# Autodesk Inventor assembly: DriveShaftA
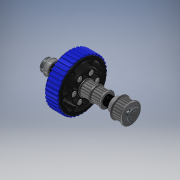
[picture p0: Inventor's stored thumbnail of the model, 180x180]
Saved by Autodesk Inventor 2018 (Build 220112000, 112)
## iProperties
Created: 2017-09-03
Part Number: DriveShaftA
Document SubType Name: Assembly
Designer: snipe
Author: snipe
## Documents named in this file (10)
- E:\Clark\Assets\DriveShaftA.iam
- E:\Clark\Assets\ThunderHex_DriveShaft.ipt
- E:\Clark\Assets\FlangedThunderHexBearing.ipt
- E:\Clark\Assets\ShaftCollar.ipt
- E:\Clark\Assets\0.5inSpacer.ipt
- E:\Clark\Assets\0.25inSpacer.ipt
- E:\Clark\Assets\0.125inSpacer.ipt
- E:\Clark\Assets\18tPulley15mm.ipt
- E:\Clark\Assets\PlactionWheelwithHubnoBearing.iam
- E:\Clark\Assets\24tPulley15mm.ipt
## Components (15 placed, 9 different names)
1. ThunderHex_DriveShaft:1 — Flush:1, Mate:1, Mate:2, Mate:4, Mate:5, Mate:7, Mate:9, Mate:10, Mate:12, Mate:13, Mate:15, Mate:16, Mate:18, Mate:19, Mate:21, Mate:22, Mate:24, Mate:25, Mate:27, Mate:28, Mate:30, Mate:32, Mate:33, Mate:35, Mate:36, Mate:38, Mate:39
2. FlangedThunderHexBearing:1 — Mate:29, Mate:30, Mate:31
3. FlangedThunderHexBearing:2 — Mate:6, Mate:7, Mate:8
4. ShaftCollar:1 — Flush:1, Mate:1, Mate:2, Mate:3
5. ShaftCollar:2 — Mate:35, Mate:36, Mate:40
6. 0.5inSpacer:1 — Mate:8, Mate:9, Mate:10, Mate:11
7. 0.5inSpacer:2 — Mate:23, Mate:24, Mate:25, Mate:26
8. 0.25inSpacer:1 — Mate:11, Mate:12, Mate:13, Mate:14
9. 0.125inSpacer:1 — Mate:26, Mate:27, Mate:28, Mate:29
10. 0.125inSpacer:2 — Mate:31, Mate:32, Mate:33, Mate:37
11. 0.125inSpacer:3 — Mate:3, Mate:4, Mate:5, Mate:6
12. 18tPulley15mm:1 — Mate:17, Mate:18, Mate:19, Mate:20
13. 18tPulley15mm:2 — Mate:20, Mate:21, Mate:22, Mate:23
14. PlactionWheelwithHubnoBearing:1 [sub-assembly] — Mate:14, Mate:15, Mate:16, Mate:17
15. 24tPulley15mm:1 — Mate:37, Mate:38, Mate:39, Mate:40
## Relationships (40: Mate 39, Flush 1)
- Flush:1: ThunderHex_DriveShaft:1 ↔ ShaftCollar:1
- Mate:1: ThunderHex_DriveShaft:1 ↔ ShaftCollar:1
- Mate:2: ThunderHex_DriveShaft:1 ↔ ShaftCollar:1
- Mate:3: ShaftCollar:1 ↔ 0.125inSpacer:3
- Mate:4: ThunderHex_DriveShaft:1 ↔ 0.125inSpacer:3
- Mate:5: ThunderHex_DriveShaft:1 ↔ 0.125inSpacer:3
- Mate:6: FlangedThunderHexBearing:2 ↔ 0.125inSpacer:3
- Mate:7: ThunderHex_DriveShaft:1 ↔ FlangedThunderHexBearing:2
- Mate:8: FlangedThunderHexBearing:2 ↔ 0.5inSpacer:1
- Mate:9: ThunderHex_DriveShaft:1 ↔ 0.5inSpacer:1
- Mate:10: ThunderHex_DriveShaft:1 ↔ 0.5inSpacer:1
- Mate:11: 0.5inSpacer:1 ↔ 0.25inSpacer:1
- Mate:12: ThunderHex_DriveShaft:1 ↔ 0.25inSpacer:1
- Mate:13: ThunderHex_DriveShaft:1 ↔ 0.25inSpacer:1
- Mate:14: 0.25inSpacer:1 ↔ PlactionWheelwithHubnoBearing:1
- Mate:15: ThunderHex_DriveShaft:1 ↔ PlactionWheelwithHubnoBearing:1
- Mate:16: ThunderHex_DriveShaft:1 ↔ PlactionWheelwithHubnoBearing:1
- Mate:17: 18tPulley15mm:1 ↔ PlactionWheelwithHubnoBearing:1
- Mate:18: ThunderHex_DriveShaft:1 ↔ 18tPulley15mm:1
- Mate:19: ThunderHex_DriveShaft:1 ↔ 18tPulley15mm:1
- Mate:20: 18tPulley15mm:1 ↔ 18tPulley15mm:2
- Mate:21: ThunderHex_DriveShaft:1 ↔ 18tPulley15mm:2
- Mate:22: ThunderHex_DriveShaft:1 ↔ 18tPulley15mm:2
- Mate:23: 0.5inSpacer:2 ↔ 18tPulley15mm:2
- Mate:24: ThunderHex_DriveShaft:1 ↔ 0.5inSpacer:2
- Mate:25: ThunderHex_DriveShaft:1 ↔ 0.5inSpacer:2
- Mate:26: 0.5inSpacer:2 ↔ 0.125inSpacer:1
- Mate:27: ThunderHex_DriveShaft:1 ↔ 0.125inSpacer:1
- Mate:28: ThunderHex_DriveShaft:1 ↔ 0.125inSpacer:1
- Mate:29: FlangedThunderHexBearing:1 ↔ 0.125inSpacer:1
- Mate:30: ThunderHex_DriveShaft:1 ↔ FlangedThunderHexBearing:1
- Mate:31: FlangedThunderHexBearing:1 ↔ 0.125inSpacer:2
- Mate:32: ThunderHex_DriveShaft:1 ↔ 0.125inSpacer:2
- Mate:33: ThunderHex_DriveShaft:1 ↔ 0.125inSpacer:2
- Mate:35: ThunderHex_DriveShaft:1 ↔ ShaftCollar:2
- Mate:36: ThunderHex_DriveShaft:1 ↔ ShaftCollar:2
- Mate:37: 0.125inSpacer:2 ↔ 24tPulley15mm:1
- Mate:38: ThunderHex_DriveShaft:1 ↔ 24tPulley15mm:1
- Mate:39: ThunderHex_DriveShaft:1 ↔ 24tPulley15mm:1
- Mate:40: ShaftCollar:2 ↔ 24tPulley15mm:1
